# Autodesk Inventor assembly: CamerCaseMountAssembly
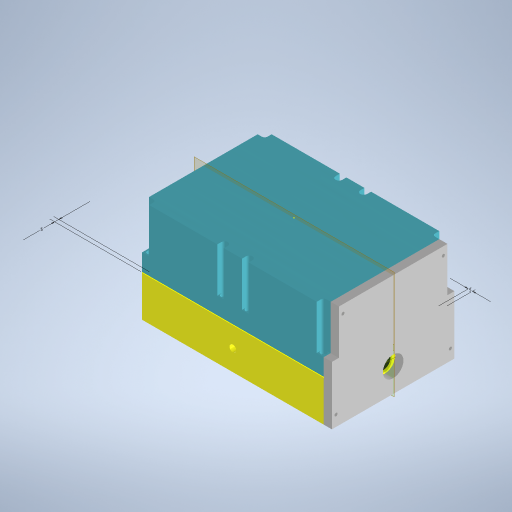
[picture p0: Inventor's stored thumbnail of the model, 512x512]
Saved by Autodesk Inventor 2023 (Build 270158030, 158C)
## iProperties
Created: 2021-08-20
Part Number: CamerCaseMountAssembly
Document SubType Name: Assembly
Designer: robst
Author: robst
## Documents named in this file (13)
- C:\git\CAD-Development\robSteele\ShapeWays\GlobalMeteorNetwork\CamerCaseMountAssembly.iam
- C:\git\CAD-Development\robSteele\ShapeWays\GlobalMeteorNetwork\caseLowerPortion.ipt
- C:\git\CAD-Development\robSteele\ShapeWays\GlobalMeteorNetwork\Raspberry Pi Canakit Case\RPI4-step.ipt
- C:\git\CAD-Development\robSteele\ShapeWays\GlobalMeteorNetwork\poeAdapter.ipt
- C:\git\CAD-Development\robSteele\ShapeWays\GlobalMeteorNetwork\IMX291 Camera Case Assembly.iam
- C:\git\CAD-Development\robSteele\ShapeWays\GlobalMeteorNetwork\caseUpperPortion.ipt
- C:\git\CAD-Development\robSteele\ShapeWays\GlobalMeteorNetwork\Fan 60x60x16.ipt
- C:\git\CAD-Development\robSteele\ShapeWays\GlobalMeteorNetwork\bracketForGarageUpperAndLowerHalfs.iam
- C:\git\CAD-Development\robSteele\Inventor2016\Content Center Files\en-US\ANSI B18.22.1\ANSI B18.22.1 - No. 10 - Type A.ipt
- C:\Users\robst\Documents\Inventor\Content Center Files\R2021\en-US\ANSI B18.3(11)\ANSI B18.3 - 10-32 UNF - 2(23).ipt
- C:\git\CAD-Development\robSteele\ShapeWays\GlobalMeteorNetwork\squareBracketForLowerGarage.ipt
- C:\git\CAD-Development\robSteele\ShapeWays\GlobalMeteorNetwork\bracketForGarageUpperMiddleAndLowerSections.iam
- C:\git\CAD-Development\robSteele\ShapeWays\GlobalMeteorNetwork\frontPlate.ipt
## Components (14 placed, 12 different names)
1. caseLowerPortion:1 — Mate:4, Mate:5, Mate:6, Mate:7, Mate:8, Mate:9, Mate:10, Mate:11, Mate:12, Mate:13, Flush:1, Flush:2, Mate:14, Mate:15, Mate:16, Insert:1, Insert:4, Insert:5, Insert:6, Mate:23, Flush:3, Flush:4
2. Fan 60x60x16:1 — Mate:14, Mate:15, Mate:16
3. RPI4-step:1 — Mate:4, Mate:5, Mate:6
4. poeAdapter:1 — Mate:7, Mate:8, Mate:9
5. IMX291 Camera Case Assembly:1 [sub-assembly] — Mate:10, Mate:11, Mate:12
6. caseUpperPortion:1 — Mate:13, Flush:1, Flush:2, Mate:17, Mate:22
7. bracketForGarageUpperAndLowerHalfs:1 [sub-assembly] — Mate:17, Insert:1, Mate:18, Mate:19, Mate:20, Mate:21
8. Plain Washer (Inch) No. 10 - Type A:1 — Mate:18, Mate:19, Insert:2
9. Spline Socket Button Head Cap Screw - Inch 10-32 UNF - 2:1 — Insert:2
10. Plain Washer (Inch) No. 10 - Type A:2 — Mate:20, Mate:21, Insert:3
11. Spline Socket Button Head Cap Screw - Inch 10-32 UNF - 2:2 — Insert:3
12. squareBracketForLowerGarage:1 — Insert:4, Insert:5
13. bracketForGarageUpperMiddleAndLowerSections:1 [sub-assembly] — Mate:22, Insert:6
14. frontPlate:1 — Mate:23, Flush:3, Flush:4
## Relationships (30: Mate 20, Insert 6, Flush 4)
- Mate:4: caseLowerPortion:1 ↔ RPI4-step:1
- Mate:5: caseLowerPortion:1 ↔ RPI4-step:1
- Mate:6: caseLowerPortion:1 ↔ RPI4-step:1
- Mate:7: caseLowerPortion:1 ↔ poeAdapter:1
- Mate:8: caseLowerPortion:1 ↔ poeAdapter:1
- Mate:9: caseLowerPortion:1 ↔ poeAdapter:1
- Mate:10: caseLowerPortion:1 ↔ IMX291 Camera Case Assembly:1
- Mate:11 (0.75 mm): caseLowerPortion:1 ↔ IMX291 Camera Case Assembly:1
- Mate:12 (0.75 mm): caseLowerPortion:1 ↔ IMX291 Camera Case Assembly:1
- Mate:13: caseLowerPortion:1 ↔ caseUpperPortion:1
- Flush:1: caseLowerPortion:1 ↔ caseUpperPortion:1
- Flush:2: caseLowerPortion:1 ↔ caseUpperPortion:1
- Mate:14: caseLowerPortion:1 ↔ Fan 60x60x16:1
- Mate:15 (1 mm): caseLowerPortion:1 ↔ Fan 60x60x16:1
- Mate:16 (0.5 mm): caseLowerPortion:1 ↔ Fan 60x60x16:1
- Mate:17: caseUpperPortion:1 ↔ bracketForGarageUpperAndLowerHalfs:1
- Insert:1 (0.5 mm): caseLowerPortion:1 ↔ bracketForGarageUpperAndLowerHalfs:1
- Mate:18: bracketForGarageUpperAndLowerHalfs:1 ↔ Plain Washer (Inch) No. 10 - Type A:1
- Mate:19: bracketForGarageUpperAndLowerHalfs:1 ↔ Plain Washer (Inch) No. 10 - Type A:1
- Mate:20: bracketForGarageUpperAndLowerHalfs:1 ↔ Plain Washer (Inch) No. 10 - Type A:2
- Mate:21: bracketForGarageUpperAndLowerHalfs:1 ↔ Plain Washer (Inch) No. 10 - Type A:2
- Insert:2: Plain Washer (Inch) No. 10 - Type A:1 ↔ Spline Socket Button Head Cap Screw - Inch 10-32 UNF - 2:1
- Insert:3: Plain Washer (Inch) No. 10 - Type A:2 ↔ Spline Socket Button Head Cap Screw - Inch 10-32 UNF - 2:2
- Insert:4: caseLowerPortion:1 ↔ squareBracketForLowerGarage:1
- Insert:5: caseLowerPortion:1 ↔ squareBracketForLowerGarage:1
- Mate:22: caseUpperPortion:1 ↔ bracketForGarageUpperMiddleAndLowerSections:1
- Insert:6: caseLowerPortion:1 ↔ bracketForGarageUpperMiddleAndLowerSections:1
- Mate:23: caseLowerPortion:1 ↔ frontPlate:1
- Flush:3: caseLowerPortion:1 ↔ frontPlate:1
- Flush:4: caseLowerPortion:1 ↔ frontPlate:1
